# Autodesk Inventor assembly: test
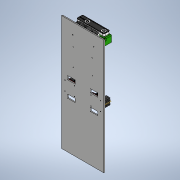
[picture p0: Inventor's stored thumbnail of the model, 180x180]
Saved by Autodesk Inventor 2020 (Build 240168000, 168)
## iProperties
Created: 2021-10-02
Part Number: test
Document SubType Name: Assembly
Designer: Петров Иван
Author: Петров Иван
## Documents named in this file (6)
- E:\IVAN\Ivan_desktop\Kvantorium\Projects\YouBotRobot\design\test_platform\test.iam
- E:\IVAN\Ivan_desktop\Kvantorium\Projects\YouBotRobot\design\test_platform\bottom.ipt
- E:\IVAN\Ivan_desktop\Kvantorium\Projects\YouBotRobot\design\test_platform\realsenses_plate_v2.ipt.iam
- E:\IVAN\Ivan_desktop\Kvantorium\Projects\YouBotRobot\design\standart_components\Odroid N2\Odroid_n2.iam
- E:\IVAN\Ivan_desktop\Kvantorium\Projects\YouBotRobot\design\standart_components\L298N\L298N_V2.ipt
- realsenses_plate_v2.ipt
## Components (5 placed, 4 different names)
1. bottom:1 — Совмещение:1, Совмещение:2, Заподлицо:1, Совмещение:3, Совмещение:5, Совмещение:6, Заподлицо:3, Заподлицо:4
2. realsenses_plate_v2.ipt:1 [sub-assembly] — Совмещение:1, Совмещение:2, Заподлицо:1, Совмещение:4, Заподлицо:2
3. Odroid_n2:1 [sub-assembly] — Совмещение:3, Совмещение:4, Заподлицо:2, Совмещение:7
4. L298N_V2:1 — Совмещение:6, Заподлицо:4, Заподлицо:5
5. L298N_V2:2 — Совмещение:5, Заподлицо:3, Заподлицо:5, Совмещение:7
## Relationships (12: Mate 7, Flush 5)
- Совмещение:1 [Mate]: bottom:1 ↔ realsenses_plate_v2.ipt:1
- Совмещение:2 [Mate]: bottom:1 ↔ realsenses_plate_v2.ipt:1
- Заподлицо:1 [Flush] (10 mm): bottom:1 ↔ realsenses_plate_v2.ipt:1
- Совмещение:3 [Mate]: bottom:1 ↔ Odroid_n2:1
- Совмещение:4 [Mate] (20 mm): realsenses_plate_v2.ipt:1 ↔ Odroid_n2:1
- Заподлицо:2 [Flush] (7.5 mm): realsenses_plate_v2.ipt:1 ↔ Odroid_n2:1
- Совмещение:5 [Mate] (5 mm): bottom:1 ↔ L298N_V2:2
- Совмещение:6 [Mate] (5 mm): bottom:1 ↔ L298N_V2:1
- Заподлицо:3 [Flush] (10 mm): bottom:1 ↔ L298N_V2:2
- Заподлицо:4 [Flush] (10 mm): bottom:1 ↔ L298N_V2:1
- Заподлицо:5 [Flush]: L298N_V2:1 ↔ L298N_V2:2
- Совмещение:7 [Mate] (50 mm): Odroid_n2:1 ↔ L298N_V2:2
